# Autodesk Inventor assembly: Default Motor Testbench Mk2
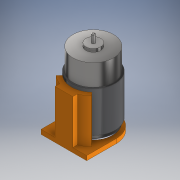
[picture p0: Inventor's stored thumbnail of the model, 180x180]
Saved by Autodesk Inventor 2018 (Build 220112000, 112)
## iProperties
Created: 2018-01-11
Part Number: Default Motor Testbench Mk2
Document SubType Name: Assembly
Designer: Moochster
Author: Moochster
## Documents named in this file (3)
- C:\Users\Moochster\OneDrive\Documents\2018 UBC\ELEC 391\Controller\CAD\Default Motor Testbench Mk2.iam
- C:\Users\Moochster\OneDrive\Documents\2018 UBC\ELEC 391\Controller\CAD\JD5B-2655W-R.ipt
- C:\Users\Moochster\OneDrive\Documents\2018 UBC\ELEC 391\Controller\CAD\Motor Face Mount.ipt
## Components (2 placed, 2 different names)
1. JD5B-2655W-R:1 — Mate:1, Mate:4
2. Motor Face Mount:1 — Mate:1, Mate:2, Mate:3, Mate:4
## Relationships (4: Mate 4)
- Mate:1: JD5B-2655W-R:1 ↔ Motor Face Mount:1
- Mate:2: Motor Face Mount:1
- Mate:3: Motor Face Mount:1
- Mate:4: JD5B-2655W-R:1 ↔ Motor Face Mount:1
